# Autodesk Inventor assembly: Side Pulley Assembly Config 1
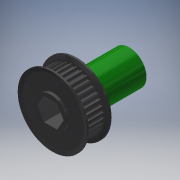
[picture p0: Inventor's stored thumbnail of the model, 180x180]
Saved by Autodesk Inventor 2018 (Build 220112000, 112)
## iProperties
Created: 2018-12-20
Part Number: Side Pulley Assembly Config 1
Document SubType Name: Assembly
Designer: maste
Author: maste
## Documents named in this file (4)
- F:\Summer Drive Base V1\Summer Drivebase\Side Pulley Assembly Config 1.iam
- F:\Summer Drive Base V1\Summer Drivebase\0.125in Spacer.ipt
- F:\Summer Drive Base V1\Summer Drivebase\1in Spacer.ipt
- F:\Summer Drive Base V1\Summer Drivebase\36t_x_9mm_Wide_Double_Flange_Aluminum_Pulley_GT2_3mm_1_2_Hex_Bore_217-5873.ipt
## Components (3 placed, 3 different names)
1. 0.125in Spacer:2 — Mate:2, Flush:3, Flush:4, Mate:3, Flush:5, Flush:6
2. 1in Spacer:1 — Mate:3, Flush:5, Flush:6
3. 36t_x_9mm_Wide_Double_Flange_Aluminum_Pulley_GT2_3mm_1_2_Hex_Bore_217-5873:1 — Mate:2, Flush:3, Flush:4
## Relationships (6: Flush 4, Mate 2)
- Mate:2: 0.125in Spacer:2 ↔ 36t_x_9mm_Wide_Double_Flange_Aluminum_Pulley_GT2_3mm_1_2_Hex_Bore_217-5873:1
- Flush:3: 0.125in Spacer:2 ↔ 36t_x_9mm_Wide_Double_Flange_Aluminum_Pulley_GT2_3mm_1_2_Hex_Bore_217-5873:1
- Flush:4: 0.125in Spacer:2 ↔ 36t_x_9mm_Wide_Double_Flange_Aluminum_Pulley_GT2_3mm_1_2_Hex_Bore_217-5873:1
- Mate:3: 0.125in Spacer:2 ↔ 1in Spacer:1
- Flush:5: 0.125in Spacer:2 ↔ 1in Spacer:1
- Flush:6: 0.125in Spacer:2 ↔ 1in Spacer:1
